# Autodesk Inventor assembly: Inner
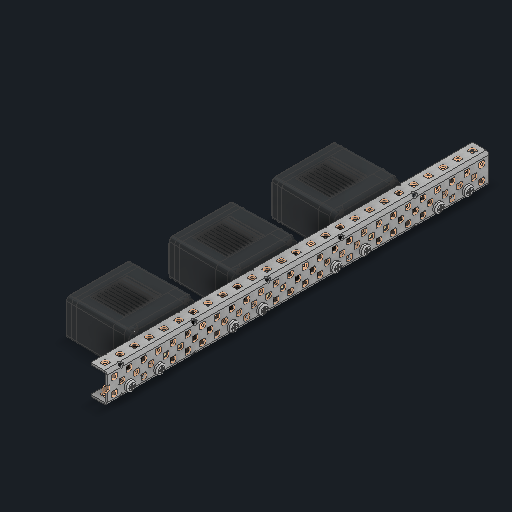
[picture p0: Inventor's stored thumbnail of the model, 512x512]
Saved by Autodesk Inventor 2025.1 (Build 291241000, 241)
## iProperties
Created: 2024-12-17
Part Number: Inner
Document SubType Name: Assembly
Designer: avere
Author: Averey Ku
## Documents named in this file (7)
- C:\Users\avere\VEX\High Stakes\CAD\V4\Chassis\Drivebay Right\Inner.iam
- C:\Users\avere\VEX\High Stakes\CAD\V4\Chassis\Drivebay Right\Alu C 1x2x1x26.ipt
- C:\Users\avere\VEX\High Stakes\CAD\V4\Chassis\Drivebay Right\Nylon Standoff .875.ipt
- C:\Users\avere\VEX\High Stakes\CAD\V4\Chassis\Drivebay Right\V5 Motor.ipt
- C:\Users\avere\VEX\High Stakes\CAD\V4\Chassis\Drivebay Right\NScrew Pan Head Threaded .500.ipt
- C:\Users\avere\VEX\High Stakes\CAD\V4\Chassis\Drivebay Right\Nut Nylon Thread-Forming.ipt
- C:\Users\avere\VEX\High Stakes\CAD\V4\Chassis\Drivebay Right\Bearing Flat Low Profile.ipt
## Components (25 placed, 6 different names)
1. Alu C 1x2x1x26:1 — Flush:3, Flush:2, Flush:1, Insert:1, Insert:10, Mate:3, Mate:2, Insert:7
2. Nylon Standoff .875:1 — Insert:1
3. V5 Motor:1 — Mate:2, Insert:7
4. V5 Motor:2
5. V5 Motor:3
6. NScrew Pan Head Threaded .500:1 — Mate:3, Insert:9
7. NScrew Pan Head Threaded .500:2 — Insert:10, Insert:8
8. Nut Nylon Thread-Forming:1 — Insert:3
9. Nut Nylon Thread-Forming:2 — Insert:2
10. Bearing Flat Low Profile:1 — Insert:2, Insert:3, Insert:8, Insert:9
11. NScrew Pan Head Threaded .500:3
12. NScrew Pan Head Threaded .500:4
13. Nut Nylon Thread-Forming:3
14. Nut Nylon Thread-Forming:4
15. Bearing Flat Low Profile:2
16. NScrew Pan Head Threaded .500:5
17. NScrew Pan Head Threaded .500:6
18. Nut Nylon Thread-Forming:5
19. Nut Nylon Thread-Forming:6
20. Bearing Flat Low Profile:3
21. NScrew Pan Head Threaded .500:7
22. NScrew Pan Head Threaded .500:8
23. Nut Nylon Thread-Forming:7
24. Nut Nylon Thread-Forming:8
25. Bearing Flat Low Profile:4
## Component patterns: (3 elements, first: V5 Motor:1), (4 elements, first: NScrew Pan Head Threaded .500:1 + NScrew Pan Head Threaded .500:2 + Nut Nylon Thread-Forming:1 + Nut Nylon Thread-Forming:2 + Bearing Flat Low Profile:1)
## Relationships (12: Insert 7, Mate 3, Flush 2)
- Flush:3 (-12.7 mm): Alu C 1x2x1x26:1
- Flush:2 (-7.9375 mm): Alu C 1x2x1x26:1
- Flush:1 [Mate] (-165.1 mm): Alu C 1x2x1x26:1
- Insert:1: Alu C 1x2x1x26:1 ↔ Nylon Standoff .875:1
- Insert:2 (1.27 mm): Nut Nylon Thread-Forming:2 ↔ Bearing Flat Low Profile:1
- Insert:3 (1.27 mm): Nut Nylon Thread-Forming:1 ↔ Bearing Flat Low Profile:1
- Insert:10: Alu C 1x2x1x26:1 ↔ NScrew Pan Head Threaded .500:2
- Insert:8 (1.5875 mm): NScrew Pan Head Threaded .500:2 ↔ Bearing Flat Low Profile:1
- Mate:3: Alu C 1x2x1x26:1 ↔ NScrew Pan Head Threaded .500:1
- Insert:9 (1.5875 mm): NScrew Pan Head Threaded .500:1 ↔ Bearing Flat Low Profile:1
- Mate:2: Alu C 1x2x1x26:1 ↔ V5 Motor:1
- Insert:7: Alu C 1x2x1x26:1 ↔ V5 Motor:1
